# Autodesk Inventor assembly: Herm
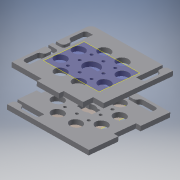
[picture p0: Inventor's stored thumbnail of the model, 180x180]
Saved by Autodesk Inventor 2016 SP1 (Build 200210100, 210)
## iProperties
Created: 2016-02-29
Part Number: Herm
Document SubType Name: Assembly
Designer: Rodrigo
Author: Rodrigo
## Documents named in this file (3)
- C:\Users\Rodrigo\Documents\2015-I\Tesis\Module\Herm.iam
- C:\Users\Rodrigo\Documents\2015-I\Tesis\Module\BottomRotated.ipt
- C:\Users\Rodrigo\Documents\2015-I\Tesis\Module\SideRotated.ipt
## Components (2 placed, 2 different names)
1. BottomRotated:1 — Mate:1, Mate:4, Mate:5
2. SideRotated:1 — Mate:1, Mate:4, Mate:5
## Relationships (3: Mate 3)
- Mate:1 (20 mm): BottomRotated:1 ↔ SideRotated:1
- Mate:4: BottomRotated:1 ↔ SideRotated:1
- Mate:5: BottomRotated:1 ↔ SideRotated:1
